# Autodesk Inventor assembly: BielaArticuladaEquipada
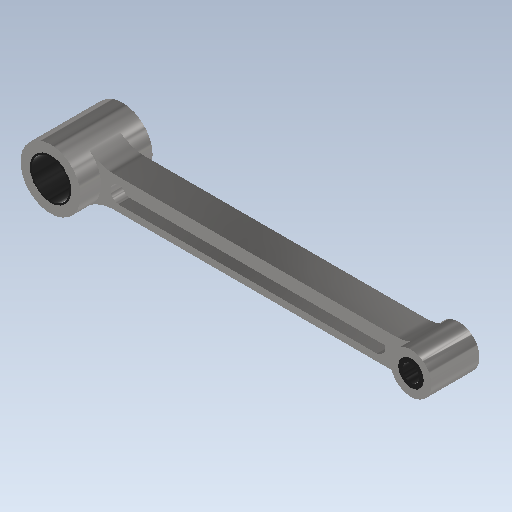
[picture p0: Inventor's stored thumbnail of the model, 512x512]
Saved by Autodesk Inventor 2021 (Build 250183000, 183)
## iProperties
Created: 2021-07-24
Part Number: BielaArticuladaEquipada
Document SubType Name: Assembly
Designer: Giovanni
Author: Giovanni
## Documents named in this file (4)
- C:\Users\irineu\Documents\Inventor\MotorRadial7\BielaArticuladaEquipada.iam
- C:\Users\irineu\Documents\Inventor\MotorRadial7\Biela Articulada.ipt
- C:\Users\irineu\Documents\Inventor\MotorRadial7\Bucha Inferior.ipt
- C:\Users\irineu\Documents\Inventor\MotorRadial7\Bucha Superior.ipt
## Components (3 placed, 3 different names)
1. Biela Articulada:1 — Inserir:1, Inserir:2
2. Bucha Inferior:1 — Inserir:2
3. Bucha Superior:1 — Inserir:1
## Relationships (2: Insert 2)
- Inserir:1: Biela Articulada:1 ↔ Bucha Superior:1
- Inserir:2: Biela Articulada:1 ↔ Bucha Inferior:1
